# Autodesk Inventor assembly: Link
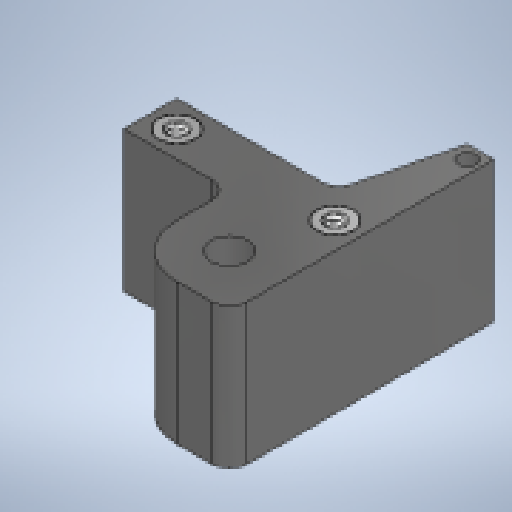
[picture p0: Inventor's stored thumbnail of the model, 512x512]
Saved by Autodesk Inventor 2023.2 (Build 272271000, 271)
## iProperties
Created: 2023-06-29
Part Number: Link
Document SubType Name: Assembly
Designer: Nathan Cai
Author: Nathan Cai
## Documents named in this file (3)
- E:\Documents\Inventor\Law - V1.0\Link.iam
- E:\Documents\Inventor\Law - V1.0\Weapon Link.ipt
- E:\Documents\Inventor\Law - V1.0\Standoff 1in.ipt
## Components (3 placed, 2 different names)
1. Weapon Link:1 — Mate:1, Mate:2, Flush:1, Flush:2
2. Standoff 1in:1 — Mate:2, Flush:2
3. Standoff 1in:2 — Mate:1, Flush:1
## Relationships (4: Mate 2, Flush 2)
- Mate:1: Weapon Link:1 ↔ Standoff 1in:2
- Mate:2: Weapon Link:1 ↔ Standoff 1in:1
- Flush:1: Weapon Link:1 ↔ Standoff 1in:2
- Flush:2: Weapon Link:1 ↔ Standoff 1in:1
